# Autodesk Inventor assembly: Shaft Collar Metal
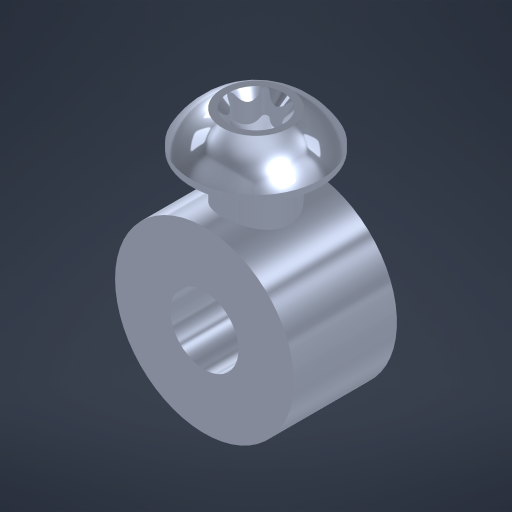
[picture p0: Inventor's stored thumbnail of the model, 512x512]
Saved by Autodesk Inventor 2023.2 (Build 272271000, 271)
## iProperties
Created: 2022-08-01
Part Number: Shaft Collar Metal
Document SubType Name: Assembly
Designer: ylu12
Author: ylu12
## Documents named in this file (5)
- D:\CAD\Parts\standard\Motion\Shafts\Shaft Collar\Shaft Collar Star Smooth.iam
- D:\CAD\Parts\standard\Motion\Shafts\Reference Parts\Shaft Collar Metal.ipt
- D:\CAD\Parts\standard\Structure\Connectors\Screw Steel - Star\SScrew Star Smooth .250.ipt
- D:\CAD\Parts\standard\Structure\Connectors\Screw Steel - Star.ipt
- D:\CAD\Parts\standard\Motion\Shafts\Shaft Collar.iam
## Components (2 placed, 2 different names)
1. Shaft Collar Metal:1 — Mate:1, Mate:2, Flush:1, Insert:4
2. SScrew Star Smooth .250:2 — Insert:4
## Relationships (4: Mate 2, Flush 1, Insert 1)
- Mate:1: Shaft Collar Metal:1
- Mate:2: Shaft Collar Metal:1
- Flush:1: Shaft Collar Metal:1
- Insert:4 (2.54 mm): Shaft Collar Metal:1 ↔ SScrew Star Smooth .250:2
